# Autodesk Inventor assembly: Assembly1
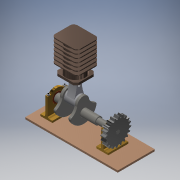
[picture p0: Inventor's stored thumbnail of the model, 180x180]
Saved by Autodesk Inventor 2019 (Build 230136000, 136)
## iProperties
Created: 2022-01-28
Part Number: Assembly1
Document SubType Name: Assembly
Designer: Sepehr
Author: Sepehr
## Documents named in this file (12)
- G:\UOK\Emtehan naghshe 2\Assembly1.iam
- G:\UOK\Emtehan naghshe 2\Part6.ipt
- G:\UOK\Emtehan naghshe 2\Part8.ipt
- G:\UOK\Emtehan naghshe 2\PartA.ipt
- G:\UOK\Emtehan naghshe 2\Part10.ipt
- G:\UOK\Emtehan naghshe 2\Part5.ipt
- G:\UOK\Emtehan naghshe 2\PartB.ipt
- G:\UOK\Emtehan naghshe 2\Part11.ipt
- G:\UOK\Emtehan naghshe 2\Part12.ipt
- G:\UOK\Emtehan naghshe 2\Part7.ipt
- G:\UOK\Emtehan naghshe 2\Part2.ipt
- G:\UOK\Emtehan naghshe 2\Part4.ipt
## Components (17 placed, 11 different names)
1. Part6:1 — Mate:1, Mate:2
2. Part8:1 — Mate:1, Insert:1, Insert:4, Mate:4, Mate:5
3. Part8:2 — Mate:2, Insert:2, Mate:3
4. PartA:1 — Insert:1, Insert:2, Insert:3, Insert:5, Insert:6
5. Part10:1 — Insert:3
6. Part10:2 — Insert:4
7. Part5:2 — Mate:3, Insert:12, Insert:13
8. Part5:3 — Mate:4, Mate:5, Insert:10, Insert:11
9. PartB:1 — Insert:5, Insert:7
10. Part11:1 — Insert:6
11. Part12:1 — Insert:7, Insert:8, Insert:9
12. Part7:1 — Insert:8
13. Part2:1 — Insert:9
14. Part4:1 — Insert:10
15. Part4:2 — Insert:11
16. Part4:3 — Insert:12
17. Part4:4 — Insert:13
## Relationships (18: Insert 13, Mate 5)
- Mate:1: Part6:1 ↔ Part8:1
- Mate:2: Part6:1 ↔ Part8:2
- Insert:1: Part8:1 ↔ PartA:1
- Insert:2: Part8:2 ↔ PartA:1
- Insert:3: PartA:1 ↔ Part10:1
- Insert:4: Part8:1 ↔ Part10:2
- Mate:3: Part8:2 ↔ Part5:2
- Mate:4: Part8:1 ↔ Part5:3
- Mate:5: Part8:1 ↔ Part5:3
- Insert:5: PartA:1 ↔ PartB:1
- Insert:6: PartA:1 ↔ Part11:1
- Insert:7: PartB:1 ↔ Part12:1
- Insert:8: Part12:1 ↔ Part7:1
- Insert:9: Part12:1 ↔ Part2:1
- Insert:10: Part5:3 ↔ Part4:1
- Insert:11: Part5:3 ↔ Part4:2
- Insert:12: Part5:2 ↔ Part4:3
- Insert:13: Part5:2 ↔ Part4:4
